# Autodesk Inventor assembly: CutHalf
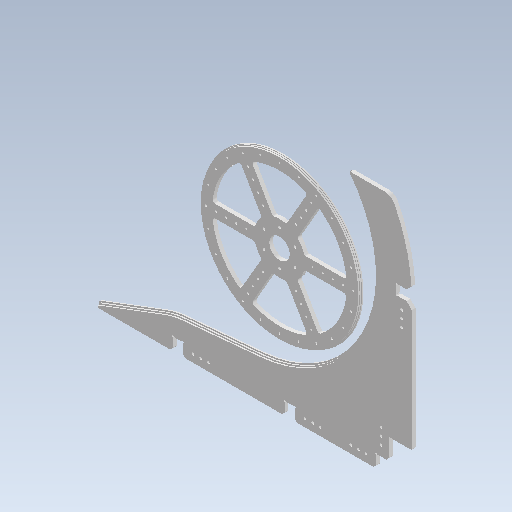
[picture p0: Inventor's stored thumbnail of the model, 512x512]
Saved by Autodesk Inventor 2020 (Build 240168000, 168)
## iProperties
Created: 2020-01-26
Part Number: CutHalf
Document SubType Name: Assembly
Designer: srini
Author: srini
## Documents named in this file (3)
- C:\Users\srini\Documents\FRC\2020\IntakeShooter\CutHalf.iam
- C:\Users\srini\Documents\FRC\2020\IntakeShooter\Ball_IndexerC.ipt
- C:\Users\srini\Documents\FRC\2020\IntakeShooter\IndexerWheelV2.ipt
## Components (2 placed, 2 different names)
1. Ball_IndexerC:1 — Flush:1, Mate:1, Mate:2
2. IndexerWheelV2:1 — Flush:1, Mate:1, Mate:2
## Relationships (3: Mate 2, Flush 1)
- Flush:1: Ball_IndexerC:1 ↔ IndexerWheelV2:1
- Mate:1 (-330.2 mm): Ball_IndexerC:1 ↔ IndexerWheelV2:1
- Mate:2 (-355.6 mm): Ball_IndexerC:1 ↔ IndexerWheelV2:1
